# Autodesk Inventor assembly: DD_KVD_003
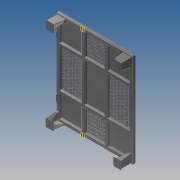
[picture p0: Inventor's stored thumbnail of the model, 180x180]
Saved by Autodesk Inventor 2017.3 (Build 213256000, 256)
## iProperties
Created: 2023-12-08
Part Number: DD_KVD_003
Document SubType Name: Weldment
Designer: Darena
Weld Material: SVAŘENEC
Author: Darena
## Documents named in this file (12)
- D:\2_Darena\1_Soukrome\02_Inventor soukromé\Dílna RAKO3\Záhora\Pivovar KONTEJNER\S výklopným dnem\DD_KVD_001\DD_KVD_003.iam
- D:\2_Darena\1_Soukrome\02_Inventor soukromé\Dílna RAKO3\Záhora\Pivovar KONTEJNER\S výklopným dnem\DD_KVD_001\DD_KVD_003_01.ipt
- D:\2_Darena\1_Soukrome\02_Inventor soukromé\Dílna RAKO3\Záhora\Pivovar KONTEJNER\S výklopným dnem\DD_KVD_001\DD_KVD_003_02.ipt
- D:\2_Darena\1_Soukrome\02_Inventor soukromé\Dílna RAKO3\Záhora\Pivovar KONTEJNER\S výklopným dnem\DD_KVD_001\DD_KVD_003_03.ipt
- D:\2_Darena\1_Soukrome\02_Inventor soukromé\Dílna RAKO3\Záhora\Pivovar KONTEJNER\S výklopným dnem\DD_KVD_001\DD_KVD_003_04.ipt
- D:\2_Darena\1_Soukrome\02_Inventor soukromé\Dílna RAKO3\Záhora\Pivovar KONTEJNER\S výklopným dnem\DD_KVD_001\DD_KVD_003_05.ipt
- D:\2_Darena\1_Soukrome\02_Inventor soukromé\Dílna RAKO3\Záhora\Pivovar KONTEJNER\S výklopným dnem\DD_KVD_001\DD_KVD_003_06.ipt
- D:\2_Darena\1_Soukrome\02_Inventor soukromé\Dílna RAKO3\Záhora\Pivovar KONTEJNER\S výklopným dnem\DD_KVD_001\DD_KVD_003_07.ipt
- D:\2_Darena\1_Soukrome\02_Inventor soukromé\Dílna RAKO3\Záhora\Pivovar KONTEJNER\S výklopným dnem\DD_KVD_001\DD_KVD_003_08.ipt
- D:\2_Darena\1_Soukrome\02_Inventor soukromé\Dílna RAKO3\Záhora\Pivovar KONTEJNER\S výklopným dnem\DD_KVD_001\DD_KVD_009.iam
- D:\2_Darena\1_Soukrome\02_Inventor soukromé\Dílna RAKO3\Záhora\Pivovar KONTEJNER\S výklopným dnem\DD_KVD_001\DD_KVD_003_10_E.ipt
- D:\2_Darena\1_Soukrome\02_Inventor soukromé\Dílna RAKO3\Záhora\Pivovar KONTEJNER\S výklopným dnem\DD_KVD_001\DD_KVD_002_14.ipt
## Components (25 placed, 11 different names)
1. DD_KVD_003_01:1 — Proti sobě:52, Proti sobě:53, Stejný směr:28, Proti sobě:65, Proti sobě:66, Proti sobě:68, Proti sobě:69, Proti sobě:71, Proti sobě:72, Proti sobě:74, Proti sobě:75, Proti sobě:76, Proti sobě:77, Proti sobě:78, Proti sobě:79, Proti sobě:80, Proti sobě:81, Proti sobě:86
2. DD_KVD_003_02:1 — Proti sobě:2, Stejný směr:4, Proti sobě:3, Proti sobě:4, Stejný směr:5, Proti sobě:5, Proti sobě:37, Proti sobě:43, Proti sobě:49, Proti sobě:52, Proti sobě:54, Stejný směr:27, Proti sobě:73, Proti sobě:83, Stejný směr:29
3. DD_KVD_003_02:2 — Proti sobě:44, Proti sobě:45, Stejný směr:24, Proti sobě:46, Proti sobě:63, Proti sobě:64, Proti sobě:84, Proti sobě:85
4. DD_KVD_003_03:1 — Proti sobě:2, Stejný směr:4, Proti sobě:3, Proti sobě:12, Proti sobě:25, Proti sobě:26, Proti sobě:42, Proti sobě:44, Proti sobě:45, Stejný směr:24, Stejný směr:25, Proti sobě:47, Stejný směr:26, Proti sobě:57, Proti sobě:70, Proti sobě:82
5. DD_KVD_003_05:1 — Stejný směr:10, Stejný směr:14, Stejný směr:15, Stejný směr:17, Stejný směr:18, Stejný směr:19, Proti sobě:26, Proti sobě:50
6. DD_KVD_003_05:2 — Stejný směr:11, Stejný směr:16, Stejný směr:19, Proti sobě:27, Proti sobě:51
7. DD_KVD_003_05:3 — Stejný směr:13, Stejný směr:16, Proti sobě:22, Proti sobě:49
8. DD_KVD_003_05:4 — Stejný směr:13, Stejný směr:14, Stejný směr:15, Proti sobě:24
9. DD_KVD_003_06:1 — Stejný směr:12, Stejný směr:17, Proti sobě:48
10. DD_KVD_003_06:2 — Proti sobě:18, Stejný směr:9, Stejný směr:11, Stejný směr:12, Proti sobě:23
11. DD_KVD_003_03:2 — Proti sobě:4, Stejný směr:5, Proti sobě:5, Proti sobě:27, Proti sobě:36, Proti sobě:38, Proti sobě:39, Proti sobě:60, Proti sobě:67
12. DD_KVD_003_04:2 — Proti sobě:22, Proti sobě:23, Proti sobě:24, Stejný směr:18, Proti sobě:25, Stejný směr:26, Proti sobě:48
13. DD_KVD_003_04:1 — Proti sobě:12, Proti sobě:18, Stejný směr:9, Stejný směr:10, Proti sobě:50, Proti sobě:51
14. DD_KVD_003_07:1 — Proti sobě:54, Proti sobě:73, Proti sobě:74, Proti sobě:75
15. DD_KVD_003_07:2 — Proti sobě:63, Proti sobě:64, Proti sobě:65, Proti sobě:66
16. DD_KVD_003_08:1 — Proti sobě:57, Proti sobě:70, Proti sobě:71, Proti sobě:72
17. DD_KVD_003_08:2 — Proti sobě:60, Proti sobě:67, Proti sobě:68, Proti sobě:69
18. DD_KVD_009:1 [sub-assembly] — Proti sobě:36, Proti sobě:37, Proti sobě:38, Stejný směr:20, Stejný směr:22
19. DD_KVD_009:2 [sub-assembly] — Proti sobě:39, Stejný směr:20, Stejný směr:21
20. DD_KVD_009:3 [sub-assembly] — Stejný směr:21, Proti sobě:42, Stejný směr:23, Proti sobě:46, Proti sobě:82
21. DD_KVD_009:4 [sub-assembly] — Proti sobě:43, Stejný směr:22, Stejný směr:23
22. DD_KVD_003_10_E:1 — Proti sobě:76, Proti sobě:77, Proti sobě:78
23. DD_KVD_003_10_E:2 — Proti sobě:79, Proti sobě:80, Proti sobě:81
24. DD_KVD_002_14:1 — Proti sobě:84, Proti sobě:85, Proti sobě:86, Proti sobě:87
25. DD_KVD_002_14:2 — Proti sobě:83, Stejný směr:29, Proti sobě:87
## Relationships (79: Mate 56, Flush 23)
- Proti sobě:2 [Mate]: DD_KVD_003_02:1 ↔ DD_KVD_003_03:1
- Stejný směr:4 [Flush]: DD_KVD_003_02:1 ↔ DD_KVD_003_03:1
- Proti sobě:3 [Mate]: DD_KVD_003_02:1 ↔ DD_KVD_003_03:1
- Proti sobě:4 [Mate]: DD_KVD_003_02:1 ↔ DD_KVD_003_03:2
- Stejný směr:5 [Flush]: DD_KVD_003_02:1 ↔ DD_KVD_003_03:2
- Proti sobě:5 [Mate]: DD_KVD_003_02:1 ↔ DD_KVD_003_03:2
- Proti sobě:12 [Mate]: DD_KVD_003_03:1 ↔ DD_KVD_003_04:1
- Proti sobě:18 [Mate]: DD_KVD_003_06:2 ↔ DD_KVD_003_04:1
- Stejný směr:9 [Flush]: DD_KVD_003_06:2 ↔ DD_KVD_003_04:1
- Stejný směr:10 [Flush]: DD_KVD_003_05:1 ↔ DD_KVD_003_04:1
- Stejný směr:11 [Flush]: DD_KVD_003_05:2 ↔ DD_KVD_003_06:2
- Stejný směr:12 [Flush]: DD_KVD_003_06:1 ↔ DD_KVD_003_06:2
- Stejný směr:13 [Flush]: DD_KVD_003_05:3 ↔ DD_KVD_003_05:4
- Stejný směr:14 [Flush]: DD_KVD_003_05:1 ↔ DD_KVD_003_05:4
- Stejný směr:15 [Flush]: DD_KVD_003_05:1 ↔ DD_KVD_003_05:4
- Stejný směr:16 [Flush]: DD_KVD_003_05:2 ↔ DD_KVD_003_05:3
- Stejný směr:17 [Flush]: DD_KVD_003_05:1 ↔ DD_KVD_003_06:1
- Proti sobě:22 [Mate]: DD_KVD_003_05:3 ↔ DD_KVD_003_04:2
- Proti sobě:23 [Mate]: DD_KVD_003_06:2 ↔ DD_KVD_003_04:2
- Proti sobě:24 [Mate]: DD_KVD_003_05:4 ↔ DD_KVD_003_04:2
- Stejný směr:18 [Flush]: DD_KVD_003_05:1 ↔ DD_KVD_003_04:2
- Proti sobě:25 [Mate]: DD_KVD_003_03:1 ↔ DD_KVD_003_04:2
- Stejný směr:19 [Flush]: DD_KVD_003_05:1 ↔ DD_KVD_003_05:2
- Proti sobě:26 [Mate] (250 mm): DD_KVD_003_03:1 ↔ DD_KVD_003_05:1
- Proti sobě:27 [Mate] (250 mm): DD_KVD_003_05:2 ↔ DD_KVD_003_03:2
- Proti sobě:36 [Mate]: DD_KVD_003_03:2 ↔ DD_KVD_009:1
- Proti sobě:37 [Mate] (3 mm): DD_KVD_003_02:1 ↔ DD_KVD_009:1
- Proti sobě:38 [Mate] (3 mm): DD_KVD_003_03:2 ↔ DD_KVD_009:1
- Proti sobě:39 [Mate]: DD_KVD_003_03:2 ↔ DD_KVD_009:2
- Stejný směr:20 [Flush]: DD_KVD_009:1 ↔ DD_KVD_009:2
- Stejný směr:21 [Flush]: DD_KVD_009:2 ↔ DD_KVD_009:3
- Proti sobě:42 [Mate] (3 mm): DD_KVD_003_03:1 ↔ DD_KVD_009:3
- Proti sobě:43 [Mate]: DD_KVD_003_02:1 ↔ DD_KVD_009:4
- Stejný směr:22 [Flush]: DD_KVD_009:1 ↔ DD_KVD_009:4
- Stejný směr:23 [Flush]: DD_KVD_009:3 ↔ DD_KVD_009:4
- Proti sobě:44 [Mate]: DD_KVD_003_02:2 ↔ DD_KVD_003_03:1
- Proti sobě:45 [Mate]: DD_KVD_003_02:2 ↔ DD_KVD_003_03:1
- Stejný směr:24 [Flush]: DD_KVD_003_02:2 ↔ DD_KVD_003_03:1
- Proti sobě:46 [Mate] (3 mm): DD_KVD_003_02:2 ↔ DD_KVD_009:3
- Stejný směr:25 [Flush]: DD_KVD_003_03:1
- Proti sobě:47 [Mate]: DD_KVD_003_03:1
- Stejný směr:26 [Flush]: DD_KVD_003_03:1 ↔ DD_KVD_003_04:2
- Proti sobě:48 [Mate]: DD_KVD_003_06:1 ↔ DD_KVD_003_04:2
- Proti sobě:49 [Mate]: DD_KVD_003_02:1 ↔ DD_KVD_003_05:3
- Proti sobě:50 [Mate]: DD_KVD_003_05:1 ↔ DD_KVD_003_04:1
- Proti sobě:51 [Mate]: DD_KVD_003_05:2 ↔ DD_KVD_003_04:1
- Proti sobě:52 [Mate]: DD_KVD_003_01:1 ↔ DD_KVD_003_02:1
- Proti sobě:53 [Mate]: DD_KVD_003_01:1
- Proti sobě:54 [Mate]: DD_KVD_003_02:1 ↔ DD_KVD_003_07:1
- Proti sobě:57 [Mate]: DD_KVD_003_03:1 ↔ DD_KVD_003_08:1
- Proti sobě:60 [Mate]: DD_KVD_003_03:2 ↔ DD_KVD_003_08:2
- Proti sobě:63 [Mate]: DD_KVD_003_02:2 ↔ DD_KVD_003_07:2
- Stejný směr:27 [Flush]: DD_KVD_003_02:1
- Stejný směr:28 [Flush]: DD_KVD_003_01:1
- Proti sobě:64 [Mate]: DD_KVD_003_02:2 ↔ DD_KVD_003_07:2
- Proti sobě:65 [Mate]: DD_KVD_003_01:1 ↔ DD_KVD_003_07:2
- Proti sobě:66 [Mate]: DD_KVD_003_01:1 ↔ DD_KVD_003_07:2
- Proti sobě:67 [Mate]: DD_KVD_003_03:2 ↔ DD_KVD_003_08:2
- Proti sobě:68 [Mate]: DD_KVD_003_01:1 ↔ DD_KVD_003_08:2
- Proti sobě:69 [Mate]: DD_KVD_003_01:1 ↔ DD_KVD_003_08:2
- Proti sobě:70 [Mate]: DD_KVD_003_03:1 ↔ DD_KVD_003_08:1
- Proti sobě:71 [Mate]: DD_KVD_003_01:1 ↔ DD_KVD_003_08:1
- Proti sobě:72 [Mate]: DD_KVD_003_01:1 ↔ DD_KVD_003_08:1
- Proti sobě:73 [Mate]: DD_KVD_003_02:1 ↔ DD_KVD_003_07:1
- Proti sobě:74 [Mate]: DD_KVD_003_01:1 ↔ DD_KVD_003_07:1
- Proti sobě:75 [Mate]: DD_KVD_003_01:1 ↔ DD_KVD_003_07:1
- Proti sobě:76 [Mate]: DD_KVD_003_01:1 ↔ DD_KVD_003_10_E:1
- Proti sobě:77 [Mate] (-254.5 mm): DD_KVD_003_01:1 ↔ DD_KVD_003_10_E:1
- Proti sobě:78 [Mate]: DD_KVD_003_01:1 ↔ DD_KVD_003_10_E:1
- Proti sobě:79 [Mate]: DD_KVD_003_01:1 ↔ DD_KVD_003_10_E:2
- Proti sobě:80 [Mate] (-254.5 mm): DD_KVD_003_01:1 ↔ DD_KVD_003_10_E:2
- Proti sobě:81 [Mate]: DD_KVD_003_01:1 ↔ DD_KVD_003_10_E:2
- Proti sobě:82 [Mate]: DD_KVD_003_03:1 ↔ DD_KVD_009:3
- Proti sobě:83 [Mate] (3 mm): DD_KVD_003_02:1 ↔ DD_KVD_002_14:2
- Stejný směr:29 [Flush] (6 mm): DD_KVD_003_02:1 ↔ DD_KVD_002_14:2
- Proti sobě:84 [Mate] (3 mm): DD_KVD_003_02:2 ↔ DD_KVD_002_14:1
- Proti sobě:85 [Mate]: DD_KVD_003_02:2 ↔ DD_KVD_002_14:1
- Proti sobě:86 [Mate] (-305 mm): DD_KVD_003_01:1 ↔ DD_KVD_002_14:1
- Proti sobě:87 [Mate]: DD_KVD_002_14:1 ↔ DD_KVD_002_14:2
